# Autodesk Inventor assembly: openlog sestava
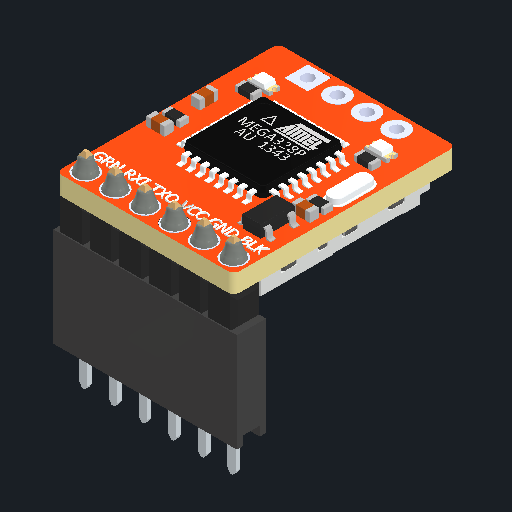
[picture p0: Inventor's stored thumbnail of the model, 512x512]
Saved by Autodesk Inventor 2022 (Build 260153000, 153)
## iProperties
Created: 2022-03-19
Part Number: openlog sestava
Document SubType Name: Assembly
Designer: dvorakj
Author: dvorakj
## Documents named in this file (3)
- C:\Users\dvorakj\Documents\Inventor\Bakalarka\Openlog\openlog sestava.iam
- C:\Users\dvorakj\Documents\Inventor\Bakalarka\Common\Header6p\header6p.iam
- C:\Users\dvorakj\Documents\Inventor\Bakalarka\Openlog\OpenLog - pins down.ipt
## Components (2 placed, 2 different names)
1. header6p:1 [sub-assembly] — Mate:1, Angle:1, Mate:2
2. OpenLog - pins down:1 — Mate:1, Angle:1, Mate:2
## Relationships (3: Mate 2, Angle 1)
- Mate:1: header6p:1 ↔ OpenLog - pins down:1
- Angle:1 (0 deg): header6p:1 ↔ OpenLog - pins down:1
- Mate:2: header6p:1 ↔ OpenLog - pins down:1
